# Autodesk Inventor assembly: backplane
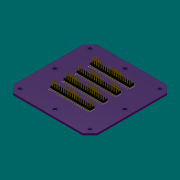
[picture p0: Inventor's stored thumbnail of the model, 180x180]
Saved by Autodesk Inventor 2016 (Build 200138000, 138)
## iProperties
Created: 2015-12-22
Part Number: backplane
Description: for SolidWorks
Document SubType Name: Assembly
Designer: sawai
Authority: Unknown
Sending System: Diptrace
Preprocessor: Open CASCADE STEP processor 6.6
Title: C:\Users\sawai\Desktop\backplane.step
Author: sawai
## Documents named in this file (3)
- C:\Users\Sawaiz\OneDrive\projects\modularRICH\frame\backplane\backplane.iam
- C:\Users\Sawaiz\OneDrive\projects\modularRICH\frame\backplane\backplanePCB.ipt
- C:\Users\Sawaiz\OneDrive\projects\modularRICH\frame\backplane\2x16header.ipt
## Components (9 placed, 2 different names)
1. backplanePCB:1 — Mate:1, Mate:2, Angle:1, Angle:5
2. 2x16header:1 — Mate:1, Flush:1, Angle:4
3. 2x16header:2 — Flush:1, Flush:2, Angle:3, Angle:4
4. 2x16header:3 — Flush:2, Flush:3, Angle:2, Angle:3
5. 2x16header:4 — Flush:3, Angle:1, Angle:2
6. 2x16header:5 — Flush:4, Angle:5, Angle:6
7. 2x16header:6 — Flush:4, Flush:5, Angle:6, Angle:7
8. 2x16header:7 — Flush:5, Flush:6, Angle:8
9. 2x16header:8 — Flush:6, Mate:2, Angle:7, Angle:8
## Relationships (16: Angle 8, Flush 6, Mate 2)
- Mate:1: backplanePCB:1 ↔ 2x16header:1
- Flush:1: 2x16header:1 ↔ 2x16header:2
- Flush:2: 2x16header:2 ↔ 2x16header:3
- Flush:3: 2x16header:3 ↔ 2x16header:4
- Flush:4: 2x16header:5 ↔ 2x16header:6
- Flush:5: 2x16header:6 ↔ 2x16header:7
- Flush:6: 2x16header:7 ↔ 2x16header:8
- Mate:2: backplanePCB:1 ↔ 2x16header:8
- Angle:1 (0 deg): backplanePCB:1 ↔ 2x16header:4
- Angle:2 (0 deg): 2x16header:3 ↔ 2x16header:4
- Angle:3 (0 deg): 2x16header:2 ↔ 2x16header:3
- Angle:4 (0 deg): 2x16header:1 ↔ 2x16header:2
- Angle:5 (0 deg): backplanePCB:1 ↔ 2x16header:5
- Angle:6 (0 deg): 2x16header:5 ↔ 2x16header:6
- Angle:7 (0 deg): 2x16header:6 ↔ 2x16header:8
- Angle:8 (0 deg): 2x16header:7 ↔ 2x16header:8
